# Autodesk Inventor assembly: SB50
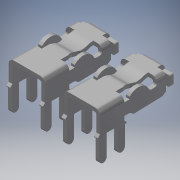
[picture p0: Inventor's stored thumbnail of the model, 180x180]
Saved by Autodesk Inventor 2019.3 (Build 233278000, 278)
## iProperties
Created: 2019-11-25
Part Number: SB50
Document SubType Name: Assembly
Designer: kjdix
Author: kjdix
## Documents named in this file (2)
- C:\Users\kjdix\Documents\EAGLE\projects\BLDC-v1\Design files\drv8353 bldc\component models\SB50.iam
- C:\Users\kjdix\Documents\EAGLE\projects\BLDC-v1\Design files\drv8353 bldc\component models\power claw.ipt
## Components (2 placed, 1 different names)
1. power claw:1 — Flush:1, Flush:2, Flush:3, Flush:4, Flush:5, Flush:6
2. power claw:2 — Flush:1, Flush:2, Flush:3
## Relationships (6: Flush 6)
- Flush:1: power claw:1 ↔ power claw:2
- Flush:2: power claw:1 ↔ power claw:2
- Flush:3 (18.415 mm): power claw:1 ↔ power claw:2
- Flush:4 (3.048 mm): power claw:1
- Flush:5: power claw:1
- Flush:6 (-3.1115 mm): power claw:1
